# Autodesk Inventor assembly: ensamblaje actuadores
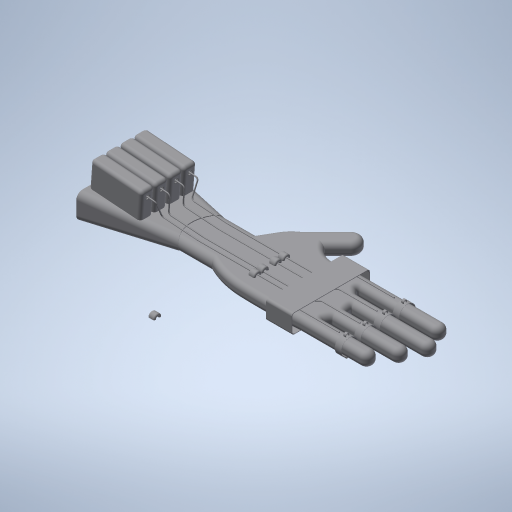
[picture p0: Inventor's stored thumbnail of the model, 512x512]
Saved by Autodesk Inventor 2023 (Build 270158000, 158)
## iProperties
Created: 2022-10-17
Part Number: ensamblaje actuadores
Document SubType Name: Assembly
Designer: Xiaba
Author: Xiaba
## Documents named in this file (13)
- C:\Users\Xiaba\Desktop\FUNBIO\Guante con actuadores\ensamblaje actuadores.iam
- C:\Users\Xiaba\Desktop\FUNBIO\Guante con actuadores\mano.ipt
- C:\Users\Xiaba\Desktop\FUNBIO\Guante con actuadores\caja de los actuadores.ipt
- C:\Users\Xiaba\Desktop\FUNBIO\Guante con actuadores\cable.ipt
- C:\Users\Xiaba\Desktop\FUNBIO\Guante con actuadores\anillos.ipt
- C:\Users\Xiaba\Desktop\FUNBIO\Guante con actuadores\cable 2.ipt
- C:\Users\Xiaba\Desktop\FUNBIO\Guante con actuadores\cable medio, anular.ipt
- C:\Users\Xiaba\Desktop\FUNBIO\Guante con actuadores\cable indice.ipt
- C:\Users\Xiaba\Desktop\FUNBIO\Guante con actuadores\cable meñique.ipt
- C:\Users\Xiaba\Desktop\FUNBIO\Guante con actuadores\cable medio.ipt
- C:\Users\Xiaba\Desktop\FUNBIO\Guante con actuadores\cable anular.ipt
- C:\Users\Xiaba\Desktop\FUNBIO\Guante con actuadores\cinta.ipt
- C:\Users\Xiaba\Desktop\FUNBIO\Guante con actuadores\seguro.ipt
## Components (31 placed, 12 different names)
1. mano:1 — Mate:1, Mate:2, Mate:3, Mate:4, Flush:1, Flush:2, Flush:3, Flush:4, Mate:9, Mate:10, Mate:11, Mate:12, Mate:48, Mate:49, Mate:50
2. caja de los actuadores:1 — Mate:1, Flush:1, Mate:8, Flush:5
3. caja de los actuadores:2 — Mate:4, Flush:3, Mate:6, Flush:7
4. caja de los actuadores:3 — Mate:2, Flush:2, Mate:7, Flush:6
5. caja de los actuadores:4 — Mate:3, Flush:4, Mate:5, Flush:8
6. cable:1 — Mate:5, Flush:8, Mate:16, Mate:17, Mate:20, Mate:21, Mate:27
7. cable:2 — Mate:6, Flush:7, Mate:22, Mate:23
8. cable:3 — Mate:7, Flush:6, Mate:24, Mate:25, Mate:26
9. cable:4 — Mate:8, Flush:5, Mate:18, Mate:19
10. anillos:1 — Mate:10, Mate:15, Mate:32
11. anillos:2 — Mate:11, Mate:15, Mate:32, Mate:33
12. anillos:3 — Mate:12, Mate:33, Mate:34
13. anillos:4 — Mate:9, Mate:34
14. cable 2:1 — Mate:16, Mate:17, Mate:20, Mate:21, Mate:27, Mate:35, Mate:36, Mate:42
15. cable 2:2 — Mate:24, Mate:25, Mate:26, Mate:30, Mate:31
16. cable 2:3 — Mate:22, Mate:23, Mate:28, Mate:29
17. cable 2:4 — Mate:18, Mate:19, Mate:37, Mate:38
18. cable medio, anular:1 — Mate:28, Mate:29, Mate:46, Mate:47
19. cable medio, anular:2 — Mate:30, Mate:31, Mate:44, Mate:45
20. cable medio, anular:3 — Mate:35, Mate:36, Mate:41, Mate:42, Mate:43
21. cable medio, anular:4 — Mate:37, Mate:38, Mate:39, Mate:40
22. cable indice:1 — Mate:39, Mate:40
23. cable meñique:1 — Mate:41, Mate:43
24. cable medio:1 — Mate:44, Mate:45
25. cable anular:1 — Mate:46, Mate:47
26. cinta:1
27. seguro:1 — Mate:49
28. seguro:2
29. seguro:3
30. seguro:4 — Mate:50
31. seguro:5 — Mate:48
## Relationships (56: Mate 48, Flush 8)
- Mate:1: mano:1 ↔ caja de los actuadores:1
- Mate:2: mano:1 ↔ caja de los actuadores:3
- Mate:3: mano:1 ↔ caja de los actuadores:4
- Mate:4: mano:1 ↔ caja de los actuadores:2
- Flush:1: mano:1 ↔ caja de los actuadores:1
- Flush:2: mano:1 ↔ caja de los actuadores:3
- Flush:3: mano:1 ↔ caja de los actuadores:2
- Flush:4: mano:1 ↔ caja de los actuadores:4
- Mate:5: caja de los actuadores:4 ↔ cable:1
- Mate:6: caja de los actuadores:2 ↔ cable:2
- Mate:7: caja de los actuadores:3 ↔ cable:3
- Mate:8: caja de los actuadores:1 ↔ cable:4
- Flush:5: caja de los actuadores:1 ↔ cable:4
- Flush:6: caja de los actuadores:3 ↔ cable:3
- Flush:7: caja de los actuadores:2 ↔ cable:2
- Flush:8: caja de los actuadores:4 ↔ cable:1
- Mate:9: mano:1 ↔ anillos:4
- Mate:10: mano:1 ↔ anillos:1
- Mate:11: mano:1 ↔ anillos:2
- Mate:12: mano:1 ↔ anillos:3
- Mate:15: anillos:1 ↔ anillos:2
- Mate:16: cable:1 ↔ cable 2:1
- Mate:17: cable:1 ↔ cable 2:1
- Mate:18: cable:4 ↔ cable 2:4
- Mate:19: cable:4 ↔ cable 2:4
- Mate:20: cable:1 ↔ cable 2:1
- Mate:21: cable:1 ↔ cable 2:1
- Mate:22: cable:2 ↔ cable 2:3
- Mate:23: cable:2 ↔ cable 2:3
- Mate:24: cable:3 ↔ cable 2:2
- Mate:25: cable:3 ↔ cable 2:2
- Mate:26: cable:3 ↔ cable 2:2
- Mate:27: cable:1 ↔ cable 2:1
- Mate:28: cable 2:3 ↔ cable medio, anular:1
- Mate:29: cable 2:3 ↔ cable medio, anular:1
- Mate:30: cable 2:2 ↔ cable medio, anular:2
- Mate:31: cable 2:2 ↔ cable medio, anular:2
- Mate:32: anillos:1 ↔ anillos:2
- Mate:33: anillos:2 ↔ anillos:3
- Mate:34: anillos:3 ↔ anillos:4
- Mate:35: cable 2:1 ↔ cable medio, anular:3
- Mate:36: cable 2:1 ↔ cable medio, anular:3
- Mate:37: cable 2:4 ↔ cable medio, anular:4
- Mate:38: cable 2:4 ↔ cable medio, anular:4
- Mate:39: cable medio, anular:4 ↔ cable indice:1
- Mate:40: cable medio, anular:4 ↔ cable indice:1
- Mate:41: cable medio, anular:3 ↔ cable meñique:1
- Mate:42: cable 2:1 ↔ cable medio, anular:3
- Mate:43: cable medio, anular:3 ↔ cable meñique:1
- Mate:44: cable medio, anular:2 ↔ cable medio:1
- Mate:45: cable medio, anular:2 ↔ cable medio:1
- Mate:46: cable medio, anular:1 ↔ cable anular:1
- Mate:47: cable medio, anular:1 ↔ cable anular:1
- Mate:48: mano:1 ↔ seguro:5
- Mate:49: mano:1 ↔ seguro:1
- Mate:50: mano:1 ↔ seguro:4
